# Autodesk Inventor assembly: Recessed Wheels V1.0
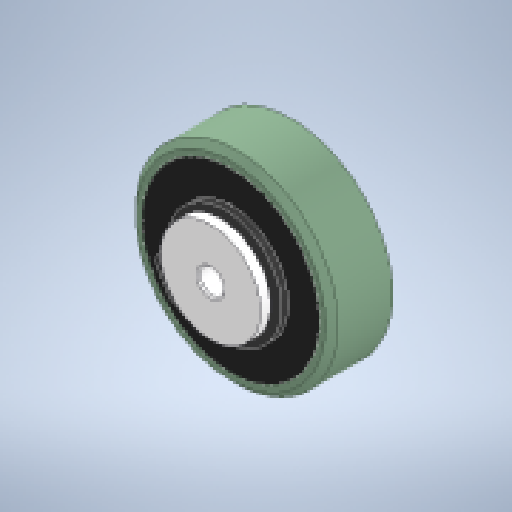
[picture p0: Inventor's stored thumbnail of the model, 512x512]
Saved by Autodesk Inventor 2023.2 (Build 272271000, 271)
## iProperties
Created: 2023-02-06
Part Number: Recessed Wheels V1.0
Document SubType Name: Assembly
Designer: Nathan Cai
Mass: 9.67901 g
Surface Area: 59.7769 cm^2
Volume: 6.59712 cm^3
Density: 1.46716 g/cm^3
Author: Nathan Cai
## Documents named in this file (4)
- C:\Users\Nathan Cai\Documents\Inventor\Flatbread V1.0\Custom Wheel V2.0\Recessed Wheels V2.0.iam
- C:\Users\Nathan Cai\Documents\Inventor\Flatbread V1.0\Custom Wheel V2.0\Tire Hub.ipt
- C:\Users\Nathan Cai\Documents\Inventor\Flatbread V1.0\Custom Wheel V2.0\Tire.ipt
- C:\Users\Nathan Cai\Documents\Inventor\Flatbread V1.0\Custom Wheel V2.0\T40_Hub_With_Retainer\T40_Hub_With_Retainer.iam
## Components (3 placed, 3 different names)
1. Tire Hub:1 — Flush:7, Mate:1, Mate:2, Mate:4
2. Tire:1 — Flush:7, Mate:1, Mate:3
3. T40_Hub_With_Retainer:1 [sub-assembly] — Mate:2, Mate:3, Mate:4
## Relationships (5: Mate 4, Flush 1)
- Flush:7: Tire Hub:1 ↔ Tire:1
- Mate:1: Tire Hub:1 ↔ Tire:1
- Mate:2 (0.0635 mm): Tire Hub:1 ↔ T40_Hub_With_Retainer:1
- Mate:3: Tire:1 ↔ T40_Hub_With_Retainer:1
- Mate:4: Tire Hub:1 ↔ T40_Hub_With_Retainer:1
